# Autodesk Inventor assembly: support assembly
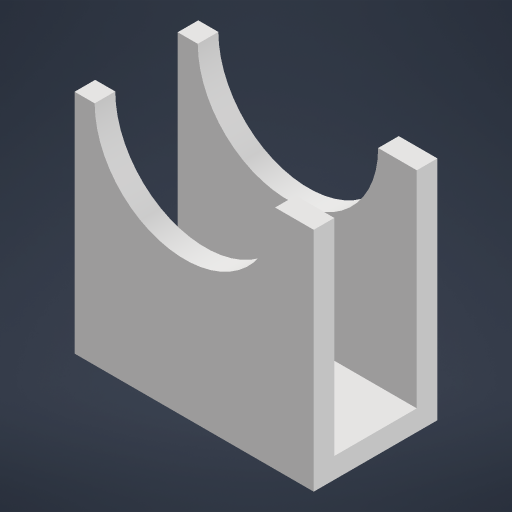
[picture p0: Inventor's stored thumbnail of the model, 512x512]
Saved by Autodesk Inventor 2023 (Build 270158000, 158)
## iProperties
Created: 2022-09-04
Part Number: support assembly
Document SubType Name: Weldment
Designer: Mike
Weld Material: Welded Aluminum-6061
Author: Mike
## Documents named in this file (3)
- C:\Users\Mike\Desktop\Mechatronics\Mechatronics 5.1\Liquid-engine-cooling-system\design files\Ethanol engine 5 -inventor files\support assembly.iam
- C:\Users\Mike\Desktop\Mechatronics\Mechatronics 5.1\Liquid-engine-cooling-system\design files\Ethanol engine 5 -inventor files\Weldedsupportpart1.ipt
- C:\Users\Mike\Desktop\Mechatronics\Mechatronics 5.1\Liquid-engine-cooling-system\design files\Ethanol engine 5 -inventor files\Weldedsupportpart2.ipt
## Components (3 placed, 2 different names)
1. Weldedsupportpart1:1 — Mate:1, Mate:2, Mate:3
2. Weldedsupportpart2:1 — Mate:1, Mate:2, Mate:3, Mate:4, Mate:5, Mate:6
3. Weldedsupportpart1:2 — Mate:4, Mate:5, Mate:6
## Relationships (6: Mate 6)
- Mate:1: Weldedsupportpart1:1 ↔ Weldedsupportpart2:1
- Mate:2: Weldedsupportpart1:1 ↔ Weldedsupportpart2:1
- Mate:3: Weldedsupportpart1:1 ↔ Weldedsupportpart2:1
- Mate:4: Weldedsupportpart2:1 ↔ Weldedsupportpart1:2
- Mate:5: Weldedsupportpart2:1 ↔ Weldedsupportpart1:2
- Mate:6: Weldedsupportpart2:1 ↔ Weldedsupportpart1:2
